# Autodesk Inventor assembly: 15x15
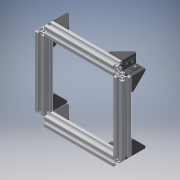
[picture p0: Inventor's stored thumbnail of the model, 180x180]
Saved by Autodesk Inventor 2016 (Build 200138000, 138)
## iProperties
Created: 2016-07-21
Part Number: 15x15
Document SubType Name: Assembly
Designer: Jonathan
Author: Jonathan
## Documents named in this file (3)
- C:\Users\Jonathan\Desktop\Models\Four Paddle Detector\frame\shapes\15x15.iam
- C:\Users\Jonathan\Desktop\Models\Four Paddle Detector\frame\extrusions\15 cm extrusion.ipt
- C:\Users\Jonathan\Desktop\Models\Four Paddle Detector\frame\brackets\angleBracket.iam
## Components (12 placed, 2 different names)
1. 15 cm extrusion:1 — Mate:9, Mate:16, Flush:14, Flush:21, Flush:27
2. 15 cm extrusion:2 — Mate:12, Mate:13, Flush:17, Flush:18, Flush:24, Flush:26
3. 15 cm extrusion:3 — Mate:14, Mate:15, Flush:15, Flush:16, Flush:25, Flush:28
4. 15 cm extrusion:4 — Mate:10, Mate:11, Flush:19, Flush:20, Flush:22, Flush:23
5. angleBracket:5 [sub-assembly] — Mate:9, Flush:21
6. angleBracket:6 [sub-assembly] — Mate:10, Flush:20, Flush:22
7. angleBracket:7 [sub-assembly] — Mate:11, Flush:19, Flush:23
8. angleBracket:8 [sub-assembly] — Mate:12, Flush:18, Flush:24
9. angleBracket:9 [sub-assembly] — Mate:13, Flush:17, Flush:26
10. angleBracket:10 [sub-assembly] — Mate:14, Flush:16, Flush:25
11. angleBracket:11 [sub-assembly] — Mate:15, Flush:15, Flush:28
12. angleBracket:12 [sub-assembly] — Mate:16, Flush:14, Flush:27
## Relationships (23: Flush 15, Mate 8)
- Mate:9: 15 cm extrusion:1 ↔ angleBracket:5
- Mate:10: 15 cm extrusion:4 ↔ angleBracket:6
- Mate:11: 15 cm extrusion:4 ↔ angleBracket:7
- Mate:12: 15 cm extrusion:2 ↔ angleBracket:8
- Mate:13: 15 cm extrusion:2 ↔ angleBracket:9
- Mate:14: 15 cm extrusion:3 ↔ angleBracket:10
- Mate:15: 15 cm extrusion:3 ↔ angleBracket:11
- Mate:16: 15 cm extrusion:1 ↔ angleBracket:12
- Flush:14: 15 cm extrusion:1 ↔ angleBracket:12
- Flush:15: 15 cm extrusion:3 ↔ angleBracket:11
- Flush:16: 15 cm extrusion:3 ↔ angleBracket:10
- Flush:17: 15 cm extrusion:2 ↔ angleBracket:9
- Flush:18: 15 cm extrusion:2 ↔ angleBracket:8
- Flush:19: 15 cm extrusion:4 ↔ angleBracket:7
- Flush:20: 15 cm extrusion:4 ↔ angleBracket:6
- Flush:21: 15 cm extrusion:1 ↔ angleBracket:5
- Flush:22: 15 cm extrusion:4 ↔ angleBracket:6
- Flush:23: 15 cm extrusion:4 ↔ angleBracket:7
- Flush:24: 15 cm extrusion:2 ↔ angleBracket:8
- Flush:25: 15 cm extrusion:3 ↔ angleBracket:10
- Flush:26: 15 cm extrusion:2 ↔ angleBracket:9
- Flush:27: 15 cm extrusion:1 ↔ angleBracket:12
- Flush:28: 15 cm extrusion:3 ↔ angleBracket:11
